# Autodesk Inventor assembly: xtion_kai
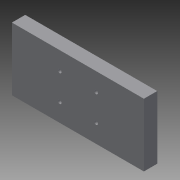
[picture p0: Inventor's stored thumbnail of the model, 180x180]
Saved by Autodesk Inventor 2013 (Build 170138000, 138)
## iProperties
Created: 2014-04-24
Part Number: xtion_kai
Document SubType Name: Assembly
Designer: andou
Author: andou
## Documents named in this file (3)
- C:\Users\andou\Documents\GitHub\Robotics-Project\design\RoboticsProject\project_4\xtion_kai.iam
- C:\Users\andou\Documents\GitHub\Robotics-Project\design\RoboticsProject\project_4\Xtion_Flame_1.ipt
- C:\Users\andou\Documents\GitHub\Robotics-Project\design\RoboticsProject\project_4\Xtion_Flame_2.ipt
## Components (2 placed, 2 different names)
1. Xtion_Flame_1:1 — フラッシュ:1, フラッシュ:2, メイト:1
2. Xtion_Flame_2:1 — フラッシュ:1, フラッシュ:2, メイト:1
## Relationships (3: Flush 2, Mate 1)
- フラッシュ:1 [Flush]: Xtion_Flame_1:1 ↔ Xtion_Flame_2:1
- フラッシュ:2 [Flush]: Xtion_Flame_1:1 ↔ Xtion_Flame_2:1
- メイト:1 [Mate]: Xtion_Flame_1:1 ↔ Xtion_Flame_2:1
